# Autodesk Inventor assembly: body_pattern
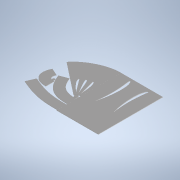
[picture p0: Inventor's stored thumbnail of the model, 180x180]
Saved by Autodesk Inventor 2020 (Build 240168000, 168)
## iProperties
Created: 2020-02-23
Part Number: body_pattern
Document SubType Name: Assembly
Designer: valem
Author: valem
## Documents named in this file (8)
- D:\Planes\Cardboard_glider_1\body_pattern.iam
- D:\Planes\Cardboard_glider_1\nose2_1.ipt
- D:\Planes\Cardboard_glider_1\nose1_1.ipt
- D:\Planes\Cardboard_glider_1\nose3_1.ipt
- D:\Planes\Cardboard_glider_1\main_body_1.ipt
- D:\Planes\Cardboard_glider_1\Tail_1.ipt
- D:\Planes\Cardboard_glider_1\nose_cone_1.ipt
- D:\Planes\Cardboard_glider_1\tail_cone_1.ipt
## Components (7 placed, 7 different names)
1. main_body_1:1 — Mate:1, Mate:8, Mate:9, Mate:10
2. nose_cone_1:1 — Mate:3
3. nose1_1:1 — Mate:5
4. nose2_1:1 — Mate:6, Mate:9
5. nose3_1:1 — Mate:7, Mate:10
6. Tail_1:1 — Mate:2, Mate:8
7. tail_cone_1:1 — Mate:4
## Relationships (10: Mate 10)
- Mate:1: main_body_1:1
- Mate:2: Tail_1:1
- Mate:3: nose_cone_1:1
- Mate:4: tail_cone_1:1
- Mate:5: nose1_1:1
- Mate:6: nose2_1:1
- Mate:7: nose3_1:1
- Mate:8: main_body_1:1 ↔ Tail_1:1
- Mate:9: main_body_1:1 ↔ nose2_1:1
- Mate:10: main_body_1:1 ↔ nose3_1:1
